# Autodesk Inventor assembly: KabineKomplett
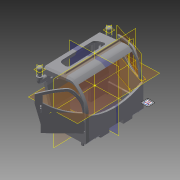
[picture p0: Inventor's stored thumbnail of the model, 180x180]
Saved by Autodesk Inventor 2015 (Build 190159000, 159)
## iProperties
Created: 2018-12-19
Part Number: KabineKomplett
Document SubType Name: Assembly
Designer: Boris
Author: Boris
## Documents named in this file (5)
- D:\Wisag Hiserv\HiSERV Smart Drive\WorkOrder\3D - Teile\KabineKomplett - Kopie.iam
- D:\Wisag Hiserv\HiSERV Smart Drive\WorkOrder\3D - Teile\KabineTeil1.ipt
- D:\Wisag Hiserv\HiSERV Smart Drive\WorkOrder\3D - Teile\KabineTürLinksRechts.ipt
- D:\Wisag Hiserv\HiSERV Smart Drive\WorkOrder\3D - Teile\KabineTürLinksRechts_MIR.ipt
- D:\Wisag Hiserv\HiSERV Smart Drive\WorkOrder\3D - Teile\Sirene.ipt
## Components (5 placed, 4 different names)
1. KabineTeil1:1 — Einfügen:1, Einfügen:5, Passend:2, Einfügen:4
2. KabineTürLinksRechts:1 — Einfügen:1
3. KabineTürLinksRechts_MIR:1 — Einfügen:4
4. Sirene:1 — Einfügen:5
5. Sirene:2 — Passend:2
## Relationships (4: Insert 3, Mate 1)
- Einfügen:1 [Insert] (-3 mm): KabineTeil1:1 ↔ KabineTürLinksRechts:1
- Einfügen:5 [Insert] (5 mm): KabineTeil1:1 ↔ Sirene:1
- Passend:2 [Mate]: KabineTeil1:1 ↔ Sirene:2
- Einfügen:4 [Insert]: KabineTeil1:1 ↔ KabineTürLinksRechts_MIR:1
